# Autodesk Inventor assembly: _Full_Ass_
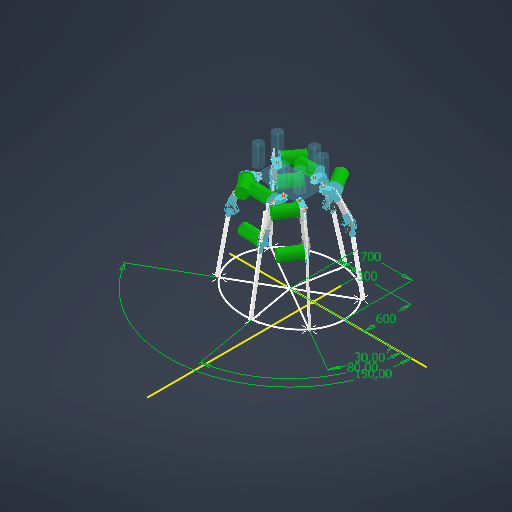
[picture p0: Inventor's stored thumbnail of the model, 512x512]
Saved by Autodesk Inventor 2026 (Build 300175000, 175)
## iProperties
RuleStatus: InUse
Created: 2026-04-24
Part Number: _Full_Ass_
Document SubType Name: Assembly
Designer: user
Mass: 69175.7 g
Surface Area: 64715.7 cm^2
Volume: 39497.9 cm^3
Density: 1.75138 g/cm^3
Author: user
## Documents named in this file (6)
- C:\Users\user\vs_code_projects\ogonek-spider\physical-structure\cad\_Full_Ass_.iam
- C:\Users\user\vs_code_projects\ogonek-spider\physical-structure\cad\leg_Left_ass.iam
- C:\Users\user\vs_code_projects\ogonek-spider\physical-structure\cad\body_frame.iam
- C:\Users\user\vs_code_projects\ogonek-spider\physical-structure\cad\leg_Right_ass.iam
- C:\Users\user\vs_code_projects\ogonek-spider\physical-structure\cad\body_parts\ground.ipt
- C:\Users\user\vs_code_projects\ogonek-spider\physical-structure\cad\parametres.xlsx
## Components (8 placed, 4 different names)
1. body_frame:1 [sub-assembly] — Заподлицо:1, С поворотом:1, С поворотом:2, С поворотом:3, С поворотом:4, С поворотом:5, С поворотом:6, Совмещение:5, Совмещение:6
2. leg_Left_ass:1 [sub-assembly] — С поворотом:2, Шаровой:7
3. leg_Left_ass:2 [sub-assembly] — С поворотом:3, Шаровой:4
4. leg_Left_ass:3 [sub-assembly] — С поворотом:1, Шаровой:3
5. leg_Right_ass:1 [sub-assembly] — С поворотом:4, Шаровой:1
6. leg_Right_ass:2 [sub-assembly] — С поворотом:5, Шаровой:2
7. leg_Right_ass:3 [sub-assembly] — С поворотом:6, Шаровой:6
8. ground:1 — Совмещение:3, Совмещение:4, Заподлицо:2, Шаровой:1, Шаровой:2, Шаровой:3, Шаровой:4, Шаровой:6, Шаровой:7
## Relationships (18: RevoluteJoint 6, BallJoint 6, Mate 4, Flush 2)
- Заподлицо:1 [Flush]: body_frame:1
- С поворотом:1 [RevoluteJoint]: body_frame:1 ↔ leg_Left_ass:3
- С поворотом:2 [RevoluteJoint]: body_frame:1 ↔ leg_Left_ass:1
- С поворотом:3 [RevoluteJoint] (50 mm): body_frame:1 ↔ leg_Left_ass:2
- С поворотом:4 [RevoluteJoint]: body_frame:1 ↔ leg_Right_ass:1
- С поворотом:5 [RevoluteJoint] (50 mm): body_frame:1 ↔ leg_Right_ass:2
- С поворотом:6 [RevoluteJoint]: body_frame:1 ↔ leg_Right_ass:3
- Совмещение:3 [Mate]: ground:1
- Совмещение:4 [Mate]: ground:1
- Совмещение:5 [Mate]: body_frame:1
- Совмещение:6 [Mate] (500 mm): body_frame:1
- Заподлицо:2 [Flush]: ground:1
- Шаровой:1 [BallJoint]: leg_Right_ass:1 ↔ ground:1
- Шаровой:2 [BallJoint]: leg_Right_ass:2 ↔ ground:1
- Шаровой:3 [BallJoint]: leg_Left_ass:3 ↔ ground:1
- Шаровой:4 [BallJoint]: leg_Left_ass:2 ↔ ground:1
- Шаровой:6 [BallJoint]: leg_Right_ass:3 ↔ ground:1
- Шаровой:7 [BallJoint]: leg_Left_ass:1 ↔ ground:1
## Named parameters: tolerance_plazma = 0.1 mm, thickness_steel = 3 mm, d_main_screw_holes = 6.1 mm, d_main_shaft = 15 mm, thickness_profile_tibea = 3 mm, width_profile_tibea = 20 mm, hight_profile_tibea = 40 mm, length_profile_tibia = 800 mm, length_thorn_tibia = 400 mm, width_profile_femur = 50 mm, hight_profile_femur = 50 mm, thickness_profile_femur = 3 mm, length_profile_femur = 350 mm, width_shaft_shift = 35 mm, hight_shaft_shift = 37 mm, width_flattened_surface = 12 mm, length_coxa = 100 mm, hight_coxa = 40 mm, width_coxa = 80 mm, width_body_l3 = 120 mm, offset_body_l23 = 200 mm, width_body_l1 = 100 mm, offset_body_l12 = 60 mm, width_body_l2 = 150 mm, hight_ground_clearance = 500 mm, iTrigger0 = 2
